# Autodesk Inventor assembly: Mechanical Workbench Step 1
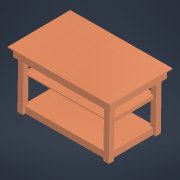
[picture p0: Inventor's stored thumbnail of the model, 180x180]
Saved by Autodesk Inventor 2022.3 (Build 263350000, 350)
## iProperties
Created: 2022-08-14
Part Number: Mechanical Workbench Step 1
Document SubType Name: Assembly
Designer: hawle
Author: hawle
## Documents named in this file (21)
- G:\Robotics 2022 CAD Files\Workshop\Mechanical Workbench Step 1.iam
- G:\Robotics 2022 CAD Files\Workshop\2x6x60 wood.ipt
- G:\Robotics 2022 CAD Files\Workshop\2x6x40_wood.ipt
- G:\Robotics 2022 CAD Files\Workshop\Mechanical Bottom.ipt
- G:\Robotics 2022 CAD Files\Workshop\3x3x42 wood.ipt
- G:\Robotics 2022 CAD Files\Workshop\2x6x72 wood.ipt
- G:\Robotics 2022 CAD Files\Workshop\2x6x33 wood.ipt
- G:\Robotics 2022 CAD Files\Workshop\2x6x44_wood.ipt
- G:\Robotics 2022 CAD Files\Workshop\Mechanical Top.ipt
- G:\Robotics 2022 CAD Files\Workshop\Mechanical Workbench Step 1\AIP\FEA\e32al848w.fins
- G:\Robotics 2022 CAD Files\Workshop\Mechanical Workbench Step 1\AIP\FEA\e32al848w.fsat
- G:\Robotics 2022 CAD Files\Workshop\Mechanical Workbench Step 1\AIP\FEA\e32al848w.ftes
- G:\Robotics 2022 CAD Files\Workshop\Mechanical Workbench Step 1\AIP\FEA\e32al848w.fwiz
- G:\Robotics 2022 CAD Files\Workshop\Mechanical Workbench Step 1\AIP\FEA\e32al849s.fins
- G:\Robotics 2022 CAD Files\Workshop\Mechanical Workbench Step 1\AIP\FEA\e32al849s.fsat
- G:\Robotics 2022 CAD Files\Workshop\Mechanical Workbench Step 1\AIP\FEA\e32al849s.ftes
- G:\Robotics 2022 CAD Files\Workshop\Mechanical Workbench Step 1\AIP\FEA\e32al849s.fwiz
- G:\Robotics 2022 CAD Files\Workshop\Mechanical Workbench Step 1\AIP\FEA\e32al84xs.fmsh
- G:\Robotics 2022 CAD Files\Workshop\Mechanical Workbench Step 1\AIP\FEA\e32al84xt.fres
- G:\Robotics 2022 CAD Files\Workshop\Mechanical Workbench Step 1\AIP\FEA\e32al85eo.fmsh
- G:\Robotics 2022 CAD Files\Workshop\Mechanical Workbench Step 1\AIP\FEA\e32al85ep.fres
## Components (20 placed, 8 different names)
1. 2x6x60 wood:1 — Flush:111, Mate:123, Flush:118
2. 2x6x60 wood:2 — Flush:114, Mate:121, Mate:122, Flush:116
3. 2x6x40_wood:1 — Flush:109, Mate:120
4. 2x6x40_wood:2 — Mate:117, Flush:110, Flush:117, Mate:124
5. Mechanical Bottom:1 — Mate:117, Flush:109, Flush:110, Flush:111, Mate:125
6. Mechanical Bottom:2 — Flush:121, Flush:122, Flush:123, Flush:124, Mate:126, Mate:127
7. 2x6x40_wood:3 — Flush:121, Flush:122
8. 2x6x40_wood:4 — Flush:123, Flush:124, Mate:125
9. 3x3x42 wood:1 — Flush:115, Mate:122, Flush:116
10. 3x3x42 wood:2 — Mate:123, Flush:117, Mate:124, Flush:119
11. 3x3x42 wood:3 — Mate:120, Flush:114, Mate:121, Flush:115, Flush:120, Mate:126, Mate:127
12. 3x3x42 wood:4 — Flush:118, Flush:119, Flush:120, Mate:137, Mate:138, Mate:139
13. 2x6x72 wood:1 — Mate:136, Mate:137
14. 2x6x72 wood:2
15. 2x6x33 wood:1
16. 2x6x33 wood:2
17. 2x6x44_wood:1 — Mate:136
18. 2x6x44_wood:2
19. 2x6x44_wood:3 — Mate:138
20. Mechanical Top:1 — Mate:139
## Relationships (51: Flush 28, Mate 23)
- Mate:117: 2x6x40_wood:2 ↔ Mechanical Bottom:1
- Flush:109: 2x6x40_wood:1 ↔ Mechanical Bottom:1
- Flush:110: 2x6x40_wood:2 ↔ Mechanical Bottom:1
- Flush:111: 2x6x60 wood:1 ↔ Mechanical Bottom:1
- [Mate]: Mechanical Bottom:2 ↔ 2x6x40_wood:4
- [Flush]: Mechanical Bottom:2 ↔ 2x6x40_wood:4
- [Mate]: Mechanical Bottom:2 ↔ 2x6x40_wood:3
- [Flush]: Mechanical Bottom:2 ↔ 2x6x40_wood:3
- Mate:120: 2x6x40_wood:1 ↔ 3x3x42 wood:3
- Flush:114: 2x6x60 wood:2 ↔ 3x3x42 wood:3
- Mate:121: 2x6x60 wood:2 ↔ 3x3x42 wood:3
- Flush:115: 3x3x42 wood:1 ↔ 3x3x42 wood:3
- Mate:122: 2x6x60 wood:2 ↔ 3x3x42 wood:1
- Flush:116: 2x6x60 wood:2 ↔ 3x3x42 wood:1
- Mate:123: 2x6x60 wood:1 ↔ 3x3x42 wood:2
- Flush:117: 2x6x40_wood:2 ↔ 3x3x42 wood:2
- Mate:124: 2x6x40_wood:2 ↔ 3x3x42 wood:2
- Flush:118: 2x6x60 wood:1 ↔ 3x3x42 wood:4
- Flush:119: 3x3x42 wood:2 ↔ 3x3x42 wood:4
- Flush:120: 3x3x42 wood:3 ↔ 3x3x42 wood:4
- Flush:121: Mechanical Bottom:2 ↔ 2x6x40_wood:3
- Flush:122: Mechanical Bottom:2 ↔ 2x6x40_wood:3
- Flush:123: Mechanical Bottom:2 ↔ 2x6x40_wood:4
- Flush:124: Mechanical Bottom:2 ↔ 2x6x40_wood:4
- Mate:125 (469.9 mm): Mechanical Bottom:1 ↔ 2x6x40_wood:4
- Mate:126: Mechanical Bottom:2 ↔ 3x3x42 wood:3
- Mate:127: Mechanical Bottom:2 ↔ 3x3x42 wood:3
- [Mate]: 2x6x72 wood:1 ↔ 2x6x44_wood:3
- [Flush]: 2x6x72 wood:1 ↔ 2x6x44_wood:3
- [Mate]: 2x6x72 wood:1 ↔ 2x6x44_wood:2
- [Flush]: 2x6x72 wood:1 ↔ 2x6x44_wood:2
- [Flush]: 2x6x72 wood:1 ↔ 2x6x44_wood:2
- [Mate]: 2x6x33 wood:2 ↔ 2x6x44_wood:1
- [Flush]: 2x6x72 wood:1 ↔ 2x6x44_wood:1
- [Mate]: 2x6x72 wood:2 ↔ 2x6x44_wood:1
- [Flush]: 2x6x72 wood:2 ↔ 2x6x44_wood:2
- [Flush]: 2x6x72 wood:2 ↔ 2x6x44_wood:1
- [Flush] (-50.8 mm): 2x6x44_wood:2 ↔ Mechanical Top:1
- [Flush] (-50.8 mm): 2x6x72 wood:2 ↔ Mechanical Top:1
- [Mate]: 2x6x44_wood:2 ↔ Mechanical Top:1
- [Mate]: 2x6x33 wood:2 ↔ 2x6x44_wood:3
- [Flush]: 2x6x33 wood:2 ↔ 2x6x44_wood:3
- [Mate]: 2x6x33 wood:1 ↔ 2x6x44_wood:1
- [Flush]: 2x6x33 wood:1 ↔ 2x6x44_wood:1
- [Flush]: 2x6x33 wood:1 ↔ 2x6x33 wood:2
- [Mate] (482.6 mm): 2x6x72 wood:1 ↔ 2x6x33 wood:2
- [Flush]: 2x6x72 wood:1 ↔ 2x6x44_wood:3
- Mate:136: 2x6x72 wood:1 ↔ 2x6x44_wood:1
- Mate:137: 3x3x42 wood:4 ↔ 2x6x72 wood:1
- Mate:138: 3x3x42 wood:4 ↔ 2x6x44_wood:3
- Mate:139: 3x3x42 wood:4 ↔ Mechanical Top:1
## Named parameters: sa_0 = 444822, sa_1 = 44482.2, sa_2 = 44482.2, sa_3 = 4.44822e+07, sa_4 = 889644, sa_5 = 444822
note: some values were not read from the file. Shown as the stored number, unit unknown: "sa_0", "sa_1", "sa_2", "sa_3", "sa_4", "sa_5".
